# Autodesk Inventor assembly: 1inThrowPancake
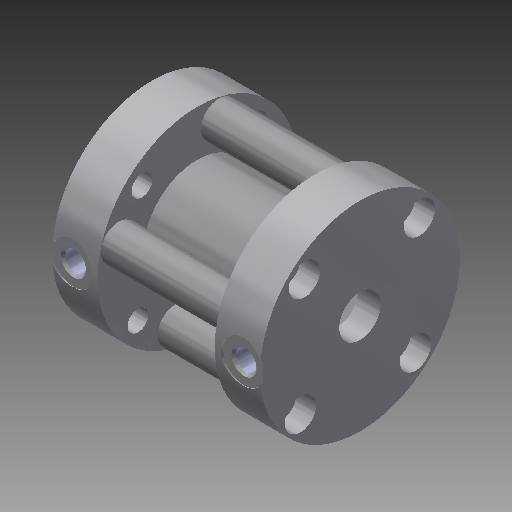
[picture p0: Inventor's stored thumbnail of the model, 512x512]
Saved by Autodesk Inventor 2017 (Build 210142000, 142)
## iProperties
Created: 2015-02-18
Part Number: 1inThrowPancake
Description: STEP AP214
Document SubType Name: Assembly
Designer: Andrew
Sending System: SolidWorks 2014
Preprocessor: SwSTEP 2.0
Title: C12010D.STEP
Revision Number: ANY
## Documents named in this file (6)
- E:\GrabCAD\2017 Robot\Gear Hanger\ActiveDrop\Parts\1inThrowPancake.iam
- E:\GrabCAD\2017 Robot\Gear Hanger\ActiveDrop\Parts\1inPancakeParts\C12010D-FO1_BM_heads.ipt
- E:\GrabCAD\2017 Robot\Gear Hanger\ActiveDrop\Parts\1inPancakeParts\C12010D-FO1_BM_tube.ipt
- E:\GrabCAD\2017 Robot\Gear Hanger\ActiveDrop\Parts\1inPancakeParts\C12010D-FO1_BM_heads (2).ipt
- E:\GrabCAD\2017 Robot\Gear Hanger\ActiveDrop\Parts\1inPancakeParts\C12010D-rod_part.ipt
- E:\GrabCAD\2017 Robot\Gear Hanger\ActiveDrop\Parts\1inPancakeParts\C12010D-FO1_BM_r.ipt
## Components (8 placed, 8 different names)
1. C12010D-FO1_BM_heads_1 — Mate:1, Mate:2, Mate:3, Mate:4, Mate:6, Mate:7, Mate:8, Mate:9, Mate:10, Mate:11, Mate:16
2. C12010D-FO1_BM_tube_2 — Mate:15, Mate:16, Mate:17
3. C12010D-FO1_BM_heads (2)_3 — Mate:14, Mate:17, Mate:18
4. C12010D-rod_part_5 — Mate:1, Mate:2, Mate:15
5. C12010D-FO1_BM_r_6 — Mate:3, Mate:4, Mate:18
6. C12010D-FO1_BM_r_7 — Mate:6, Mate:7, Mate:14
7. C12010D-FO1_BM_r_8 — Mate:10, Mate:11
8. C12010D-FO1_BM_r_9 — Mate:8, Mate:9
## Relationships (15: Mate 15)
- Mate:1: C12010D-FO1_BM_heads_1 ↔ C12010D-rod_part_5
- Mate:2: C12010D-FO1_BM_heads_1 ↔ C12010D-rod_part_5
- Mate:3: C12010D-FO1_BM_heads_1 ↔ C12010D-FO1_BM_r_6
- Mate:4: C12010D-FO1_BM_heads_1 ↔ C12010D-FO1_BM_r_6
- Mate:6: C12010D-FO1_BM_heads_1 ↔ C12010D-FO1_BM_r_7
- Mate:7: C12010D-FO1_BM_heads_1 ↔ C12010D-FO1_BM_r_7
- Mate:8: C12010D-FO1_BM_heads_1 ↔ C12010D-FO1_BM_r_9
- Mate:9: C12010D-FO1_BM_heads_1 ↔ C12010D-FO1_BM_r_9
- Mate:10: C12010D-FO1_BM_heads_1 ↔ C12010D-FO1_BM_r_8
- Mate:11: C12010D-FO1_BM_heads_1 ↔ C12010D-FO1_BM_r_8
- Mate:14: C12010D-FO1_BM_heads (2)_3 ↔ C12010D-FO1_BM_r_7
- Mate:15: C12010D-FO1_BM_tube_2 ↔ C12010D-rod_part_5
- Mate:16: C12010D-FO1_BM_heads_1 ↔ C12010D-FO1_BM_tube_2
- Mate:17: C12010D-FO1_BM_tube_2 ↔ C12010D-FO1_BM_heads (2)_3
- Mate:18: C12010D-FO1_BM_heads (2)_3 ↔ C12010D-FO1_BM_r_6
